# Autodesk Inventor assembly: ASY PRS 9100 Filter column_1200
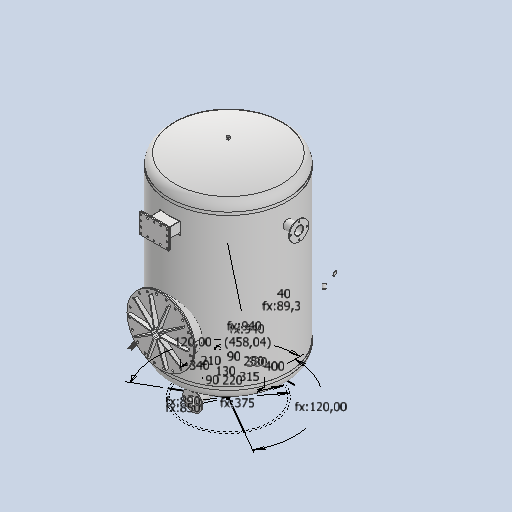
[picture p0: Inventor's stored thumbnail of the model, 512x512]
Saved by Autodesk Inventor 2026.2 (Build 302298000, 298)
## iProperties
Created: 2025-02-13
Part Number: ASY PRS 9100 Filter column_1200
Document SubType Name: Assembly
Designer: admin
Mass: 296006 g
Surface Area: 199460 cm^2
Volume: 66339.5 cm^3
Density: 4.46198 g/cm^3
Author: pokla
Revision Number: 3
## Documents named in this file (23)
- C:\Users\admin\Documents\Inventor\PRS-Purovsk\ASY PRS 1 Filter column D940_1200.iam
- C:\Users\admin\Documents\Inventor\PRS-Purovsk\PNS 9110 main Shell D 940_1200.ipt
- C:\Users\admin\Documents\Inventor\PRS-Purovsk\PNS 1604 dished head D1000_1200.ipt
- C:\Users\admin\Documents\Inventor\PRS-Purovsk\Fitting G1_1200.ipt
- C:\Users\admin\Documents\Inventor\PRS-Purovsk\PNS 1633 charging blind flange_1200.ipt
- C:\Users\admin\Documents\Inventor\PRS-Purovsk\ASY PNS 179 top funnel 1200 50-90_1000x90_1200.iam
- C:\Users\admin\Documents\Inventor\PRS-Purovsk\pallet jack dummy_1200.ipt
- C:\Users\admin\Documents\Inventor\PRS-Purovsk\ASY PNS 1610 charging hatch_1200.iam
- C:\Users\admin\Documents\Inventor\PRS-Purovsk\PNS-612 accses hatch flangeipt_1200.ipt
- C:\Users\admin\Documents\Inventor\PRS-Purovsk\PNS 1607 charging flange rect_1200.ipt
- C:\Users\admin\Documents\Inventor\PRS-Purovsk\PNS 1606 charging flange round_1200.ipt
- C:\Users\admin\Documents\Inventor\PRS-Purovsk\SLM 1671 charging tube 1_1200.ipt
- C:\Users\admin\Documents\Inventor\PRS-Purovsk\SLM 1672 charging tube 2_1200.ipt
- C:\Users\admin\Documents\Inventor\PRS-Purovsk\PNS 1615 FDS tube 5_1200.ipt
- C:\Users\admin\Documents\Inventor\PRS-Purovsk\PNS 1612 FDS tube 2_1200.ipt
- C:\Users\admin\Documents\Inventor\PRS-Purovsk\cc\JIS B 2312 90 Deg Long Elbow Steel 80A x Sch 40.ipt
- C:\Users\admin\Documents\Inventor\PRS-Purovsk\PNS-611 accses hatch tube_1200.ipt
- C:\Users\admin\Documents\Inventor\PRS-Purovsk\SLM 1432 FDS free flange DN90_1200.ipt
- C:\Users\admin\Documents\Inventor\PRS-Purovsk\SLM 1431 FDS flange DN90_1200.ipt
- C:\Users\admin\Documents\Inventor\PRS-Purovsk\PNS 1614 FDS tube 4_1200.ipt
- C:\Users\admin\Documents\Inventor\PRS-Purovsk\PNS 1613 FDS tube 3_1200.ipt
- C:\Users\admin\Documents\Inventor\PRS-Purovsk\ASY PNS 1690 Filter legs D1000_1200.iam
- C:\Users\admin\Documents\Inventor\PRS-Purovsk\ASY-PRS-DRS 940_1200.iam
## Components (27 placed, 22 different names)
1. PNS 9110 main Shell D 940_1200:1 — Flush:2, Rigid:14, Rigid:15, Rigid:16, Flush:4, Mate:1, Mate:3, Rotational:8
2. PNS 1604 dished head D1000_1200:1 — Rigid:88, Rigid:15
3. PNS 1604 dished head D1000_1200:2 — Rigid:15, Rigid:14, Mate:4
4. Fitting G1_1200:1 — Rigid:15
5. PNS 1633 charging blind flange_1200:1 — Rigid:67
6. ASY PNS 179 top funnel 1200 50-90_1000x90_1200:1 [sub-assembly] — Rotational:72
7. pallet jack dummy_1200:1
8. PNS 1633 charging blind flange_1200:2 — Rigid:77
9. PNS 1633 charging blind flange_1200:3 — Rotational:72, Rigid:78
10. ASY PNS 1610 charging hatch_1200:1 [sub-assembly] — Rotational:73
11. PNS-612 accses hatch flangeipt_1200:1 — Rotational:74, Rotational:73
12. PNS 1607 charging flange rect_1200:1 — Rigid:83
13. PNS 1606 charging flange round_1200:1 — Rigid:82, Rigid:83
14. SLM 1671 charging tube 1_1200:1 — Rigid:84
15. SLM 1672 charging tube 2_1200:1 — Rigid:84, Rigid:82, Rotational:8
16. PNS 1615 FDS tube 5_1200:1 — Rigid:73, Rigid:77, Mate:3
17. PNS 1612 FDS tube 2_1200:1 — Rigid:62, Rigid:78, Mate:4
18. JIS B 2312 90 Deg Long Elbow Steel 80A x Sch 40:1 — Rigid:62, Rigid:73
19. PNS-611 accses hatch tube_1200:1 — Rotational:74, Rigid:16
20. SLM 1432 FDS free flange DN90_1200:1 — Rigid:76, Rotational:71, Rotational:78
21. SLM 1431 FDS flange DN90_1200:1 — Rigid:76
22. PNS 1614 FDS tube 4_1200:1 — Rigid:79, Rotational:71
23. PNS 1613 FDS tube 3_1200:1 — Rigid:68, Rigid:67
24. JIS B 2312 90 Deg Long Elbow Steel 80A x Sch 40:2 — Rigid:88, Rigid:68, Rigid:79
25. Fitting G1_1200:2
26. ASY-PRS-DRS 940_1200:1 [sub-assembly] — Rotational:78
27. ASY PNS 1690 Filter legs D1000_1200:1 [sub-assembly] — Flush:5, Flush:6, Mate:2
## Relationships (30: WeldJoint 16, RevoluteJoint 6, Flush 4, Mate 4)
- Rotational:74 [RevoluteJoint]: PNS-612 accses hatch flangeipt_1200:1 ↔ PNS-611 accses hatch tube_1200:1
- Rigid:15 [WeldJoint]: PNS 1604 dished head D1000_1200:2 ↔ Fitting G1_1200:1
- Rotational:73 [RevoluteJoint]: ASY PNS 1610 charging hatch_1200:1 ↔ PNS-612 accses hatch flangeipt_1200:1
- Rigid:88 [WeldJoint]: PNS 1604 dished head D1000_1200:1 ↔ JIS B 2312 90 Deg Long Elbow Steel 80A x Sch 40:2
- Rigid:62 [WeldJoint]: PNS 1612 FDS tube 2_1200:1 ↔ JIS B 2312 90 Deg Long Elbow Steel 80A x Sch 40:1
- Rigid:68 [WeldJoint]: PNS 1613 FDS tube 3_1200:1 ↔ JIS B 2312 90 Deg Long Elbow Steel 80A x Sch 40:2
- Rigid:67 [WeldJoint]: PNS 1633 charging blind flange_1200:1 ↔ PNS 1613 FDS tube 3_1200:1
- Rigid:79 [WeldJoint]: PNS 1614 FDS tube 4_1200:1 ↔ JIS B 2312 90 Deg Long Elbow Steel 80A x Sch 40:2
- Rigid:73 [WeldJoint]: PNS 1615 FDS tube 5_1200:1 ↔ JIS B 2312 90 Deg Long Elbow Steel 80A x Sch 40:1
- Rigid:76 [WeldJoint]: SLM 1432 FDS free flange DN90_1200:1 ↔ SLM 1431 FDS flange DN90_1200:1
- Rotational:71 [RevoluteJoint]: SLM 1432 FDS free flange DN90_1200:1 ↔ PNS 1614 FDS tube 4_1200:1
- Rigid:77 [WeldJoint]: PNS 1633 charging blind flange_1200:2 ↔ PNS 1615 FDS tube 5_1200:1
- Rotational:72 [RevoluteJoint]: ASY PNS 179 top funnel 1200 50-90_1000x90_1200:1 ↔ PNS 1633 charging blind flange_1200:3
- Rigid:78 [WeldJoint]: PNS 1633 charging blind flange_1200:3 ↔ PNS 1612 FDS tube 2_1200:1
- Rigid:84 [WeldJoint]: SLM 1671 charging tube 1_1200:1 ↔ SLM 1672 charging tube 2_1200:1
- Rigid:82 [WeldJoint]: PNS 1606 charging flange round_1200:1 ↔ SLM 1672 charging tube 2_1200:1
- Rigid:83 [WeldJoint]: PNS 1607 charging flange rect_1200:1 ↔ PNS 1606 charging flange round_1200:1
- Rotational:78 [RevoluteJoint]: SLM 1432 FDS free flange DN90_1200:1 ↔ ASY-PRS-DRS 940_1200:1
- Flush:2: PNS 9110 main Shell D 940_1200:1
- Rigid:14 [WeldJoint]: PNS 9110 main Shell D 940_1200:1 ↔ PNS 1604 dished head D1000_1200:2
- Rigid:15 [WeldJoint]: PNS 9110 main Shell D 940_1200:1 ↔ PNS 1604 dished head D1000_1200:1
- Rigid:16 [WeldJoint] (20 mm): PNS 9110 main Shell D 940_1200:1 ↔ PNS-611 accses hatch tube_1200:1
- Flush:4: PNS 9110 main Shell D 940_1200:1
- Mate:1: PNS 9110 main Shell D 940_1200:1
- Flush:5: ASY PNS 1690 Filter legs D1000_1200:1
- Flush:6: ASY PNS 1690 Filter legs D1000_1200:1
- Mate:2: ASY PNS 1690 Filter legs D1000_1200:1
- Mate:3: PNS 9110 main Shell D 940_1200:1 ↔ PNS 1615 FDS tube 5_1200:1
- Mate:4: PNS 1604 dished head D1000_1200:2 ↔ PNS 1612 FDS tube 2_1200:1
- Rotational:8 [RevoluteJoint]: PNS 9110 main Shell D 940_1200:1 ↔ SLM 1672 charging tube 2_1200:1
